# Autodesk Inventor assembly: CutHalfFitTest
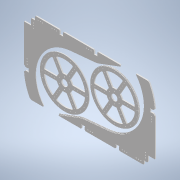
[picture p0: Inventor's stored thumbnail of the model, 180x180]
Saved by Autodesk Inventor 2020 (Build 240168000, 168)
## iProperties
Created: 2020-01-26
Part Number: CutHalfFitTest
Document SubType Name: Assembly
Designer: srini
Author: srini
## Documents named in this file (3)
- C:\Users\srini\Documents\FRC\2020\IntakeShooter\CutHalfFitTest.iam
- C:\Users\srini\Documents\FRC\2020\IntakeShooter\CutHalf.iam
- C:\Users\srini\Documents\FRC\2020\IntakeShooter\CutHalf_MIR.iam
## Components (2 placed, 2 different names)
1. CutHalf:1 [sub-assembly] — Flush:1, Mate:1, Mate:2
2. CutHalf_MIR:1 [sub-assembly] — Flush:1, Mate:1, Mate:2
## Relationships (3: Mate 2, Flush 1)
- Flush:1: CutHalf:1 ↔ CutHalf_MIR:1
- Mate:1 (-609.6 mm): CutHalf:1 ↔ CutHalf_MIR:1
- Mate:2 (-1066.8 mm): CutHalf:1 ↔ CutHalf_MIR:1
